# Autodesk Inventor assembly: POM_T5_24
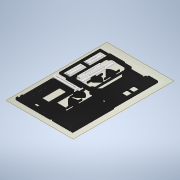
[picture p0: Inventor's stored thumbnail of the model, 180x180]
Saved by Autodesk Inventor 2020 (Build 240168000, 168)
## iProperties
Created: 2021-08-27
Part Number: POM_T5_24
Document SubType Name: Assembly
Designer: Masato
Author: Masato
## Documents named in this file (13)
- C:\Inventor\SUSTAINA-OP\Cam\POM_T5_24.iam
- C:\Inventor\SUSTAINA-OP\Cam\DisposableBoard.ipt
- C:\Inventor\SUSTAINA-OP\UpperBody\Cockpit\Cockpit_side_frame_MIR.ipt
- C:\Inventor\SUSTAINA-OP\UpperBody\Head\Camera_side_frame.ipt
- C:\Inventor\SUSTAINA-OP\UpperBody\Cockpit\Cockpit_circuit_board_frame.ipt
- C:\Inventor\SUSTAINA-OP\UpperBody\Cockpit\Cockpit_battery_back_door.ipt
- C:\Inventor\SUSTAINA-OP\UpperBody\Cockpit\Cockpit_top_frame.ipt
- C:\Inventor\SUSTAINA-OP\UpperBody\Cockpit\Cockpit_front_frame.ipt
- C:\Inventor\SUSTAINA-OP\Jig\Cockpit_battery_bottom_frame_Jig.ipt
- C:\Inventor\SUSTAINA-OP\Jig\Cockpit_front_frame_Jig.ipt
- C:\Inventor\SUSTAINA-OP\Jig\Cockpit_battery_back_door_Jig.ipt
- C:\Inventor\SUSTAINA-OP\Jig\Cockpit_carrier_board_frame_Jig.ipt
- C:\Inventor\SUSTAINA-OP\Jig\Cockpit_back_frame_Jig.ipt
## Components (15 placed, 12 different names)
1. DisposableBoard:1 — メイト:2, メイト:1, フラッシュ:1, フラッシュ:2, メイト:19, メイト:20, フラッシュ:3, フラッシュ:4, メイト:21, メイト:22, メイト:24, メイト:26, メイト:28, 角度:1, メイト:36, メイト:39, メイト:41, メイト:44, メイト:45, メイト:49, メイト:50
2. Camera_side_frame:3 — メイト:19, メイト:29, メイト:30, メイト:32
3. Cockpit_side_frame_MIR:1 — メイト:20, フラッシュ:3, フラッシュ:4, フラッシュ:5, メイト:25, フラッシュ:7, メイト:29, メイト:31, メイト:40, フラッシュ:8
4. Cockpit_circuit_board_frame:1 — メイト:28, フラッシュ:7, メイト:33, メイト:34, メイト:37, メイト:38, メイト:42, メイト:43, メイト:46, 正接:1, メイト:48, メイト:52, メイト:53
5. Cockpit_battery_back_door:1 — メイト:21, フラッシュ:6, メイト:34, メイト:35
6. Cockpit_top_frame:1 — メイト:22, メイト:27, フラッシュ:6, メイト:35
7. Cockpit_front_frame:1 — メイト:24, フラッシュ:5, メイト:25, メイト:27, メイト:30
8. Camera_side_frame:4 — メイト:26, 角度:1, メイト:31, メイト:32, メイト:33
9. Cockpit_battery_bottom_frame_Jig:1 — メイト:36, メイト:37, メイト:38
10. Cockpit_front_frame_Jig:1 — メイト:39, メイト:40, フラッシュ:8
11. Cockpit_battery_back_door_Jig:1 — メイト:41, メイト:42, メイト:43
12. Cockpit_carrier_board_frame_Jig:1 — メイト:45, メイト:47, メイト:48, メイト:51
13. Cockpit_back_frame_Jig:1 — メイト:44, メイト:46, メイト:47, 正接:1
14. Camera_side_frame:5 — メイト:49, メイト:53, 正接:2
15. Camera_side_frame:6 — メイト:50, メイト:51, メイト:52, 正接:2
## Relationships (47: Mate 36, Flush 8, Tangent 2, Angle 1)
- メイト:2 [Mate]: DisposableBoard:1
- メイト:1 [Mate]: DisposableBoard:1
- フラッシュ:1 [Flush]: DisposableBoard:1
- フラッシュ:2 [Flush]: DisposableBoard:1
- メイト:19 [Mate]: DisposableBoard:1 ↔ Camera_side_frame:3
- メイト:20 [Mate]: DisposableBoard:1 ↔ Cockpit_side_frame_MIR:1
- フラッシュ:3 [Flush] (2 mm): DisposableBoard:1 ↔ Cockpit_side_frame_MIR:1
- フラッシュ:4 [Flush] (2 mm): DisposableBoard:1 ↔ Cockpit_side_frame_MIR:1
- メイト:21 [Mate]: DisposableBoard:1 ↔ Cockpit_battery_back_door:1
- メイト:22 [Mate]: DisposableBoard:1 ↔ Cockpit_top_frame:1
- メイト:24 [Mate]: DisposableBoard:1 ↔ Cockpit_front_frame:1
- フラッシュ:5 [Flush]: Cockpit_side_frame_MIR:1 ↔ Cockpit_front_frame:1
- メイト:25 [Mate] (2.5 mm): Cockpit_side_frame_MIR:1 ↔ Cockpit_front_frame:1
- メイト:26 [Mate]: DisposableBoard:1 ↔ Camera_side_frame:4
- メイト:27 [Mate] (2.5 mm): Cockpit_top_frame:1 ↔ Cockpit_front_frame:1
- フラッシュ:6 [Flush]: Cockpit_battery_back_door:1 ↔ Cockpit_top_frame:1
- メイト:28 [Mate]: DisposableBoard:1 ↔ Cockpit_circuit_board_frame:1
- フラッシュ:7 [Flush]: Cockpit_side_frame_MIR:1 ↔ Cockpit_circuit_board_frame:1
- メイト:29 [Mate] (2.5 mm): Camera_side_frame:3 ↔ Cockpit_side_frame_MIR:1
- メイト:30 [Mate] (2.5 mm): Camera_side_frame:3 ↔ Cockpit_front_frame:1
- 角度:1 [Angle] (270 deg): DisposableBoard:1 ↔ Camera_side_frame:4
- メイト:31 [Mate] (2.5 mm): Cockpit_side_frame_MIR:1 ↔ Camera_side_frame:4
- メイト:32 [Mate] (2.5 mm): Camera_side_frame:3 ↔ Camera_side_frame:4
- メイト:33 [Mate] (2.5 mm): Cockpit_circuit_board_frame:1 ↔ Camera_side_frame:4
- メイト:34 [Mate] (2.5 mm): Cockpit_circuit_board_frame:1 ↔ Cockpit_battery_back_door:1
- メイト:35 [Mate] (2.5 mm): Cockpit_battery_back_door:1 ↔ Cockpit_top_frame:1
- メイト:36 [Mate]: DisposableBoard:1 ↔ Cockpit_battery_bottom_frame_Jig:1
- メイト:37 [Mate] (7.5 mm): Cockpit_circuit_board_frame:1 ↔ Cockpit_battery_bottom_frame_Jig:1
- メイト:38 [Mate] (5 mm): Cockpit_circuit_board_frame:1 ↔ Cockpit_battery_bottom_frame_Jig:1
- メイト:39 [Mate]: DisposableBoard:1 ↔ Cockpit_front_frame_Jig:1
- メイト:40 [Mate] (2.5 mm): Cockpit_side_frame_MIR:1 ↔ Cockpit_front_frame_Jig:1
- フラッシュ:8 [Flush]: Cockpit_side_frame_MIR:1 ↔ Cockpit_front_frame_Jig:1
- メイト:41 [Mate]: DisposableBoard:1 ↔ Cockpit_battery_back_door_Jig:1
- メイト:42 [Mate] (7.5 mm): Cockpit_circuit_board_frame:1 ↔ Cockpit_battery_back_door_Jig:1
- メイト:43 [Mate] (5.5 mm): Cockpit_circuit_board_frame:1 ↔ Cockpit_battery_back_door_Jig:1
- メイト:44 [Mate]: DisposableBoard:1 ↔ Cockpit_back_frame_Jig:1
- メイト:45 [Mate]: DisposableBoard:1 ↔ Cockpit_carrier_board_frame_Jig:1
- メイト:46 [Mate] (2.5 mm): Cockpit_circuit_board_frame:1 ↔ Cockpit_back_frame_Jig:1
- メイト:47 [Mate] (2.5 mm): Cockpit_carrier_board_frame_Jig:1 ↔ Cockpit_back_frame_Jig:1
- 正接:1 [Tangent] (2.5 mm): Cockpit_circuit_board_frame:1 ↔ Cockpit_back_frame_Jig:1
- メイト:48 [Mate] (2.5 mm): Cockpit_circuit_board_frame:1 ↔ Cockpit_carrier_board_frame_Jig:1
- メイト:49 [Mate]: DisposableBoard:1 ↔ Camera_side_frame:5
- メイト:50 [Mate]: DisposableBoard:1 ↔ Camera_side_frame:6
- メイト:51 [Mate] (2.5 mm): Cockpit_carrier_board_frame_Jig:1 ↔ Camera_side_frame:6
- メイト:52 [Mate] (9.5 mm): Cockpit_circuit_board_frame:1 ↔ Camera_side_frame:6
- メイト:53 [Mate] (2.5 mm): Cockpit_circuit_board_frame:1 ↔ Camera_side_frame:5
- 正接:2 [Tangent] (2.5 mm): Camera_side_frame:5 ↔ Camera_side_frame:6
